# Autodesk Inventor assembly: AviBay
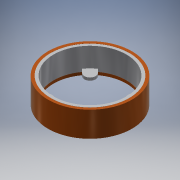
[picture p0: Inventor's stored thumbnail of the model, 180x180]
Saved by Autodesk Inventor 2017 (Build 210142000, 142)
## iProperties
Created: 2016-10-18
Part Number: AviBay
Document SubType Name: Assembly
Designer: cflannery
Author: cflannery
## Documents named in this file (3)
- D:\Triton_Rocket_Club\Propulsion\Launches\8-inch-flight\Design\CAD\Other\AviBay\trunk\AviBay.iam
- D:\Triton_Rocket_Club\Propulsion\Launches\8-inch-flight\Design\CAD\Other\AviBay\trunk\aluminumMount.ipt
- D:\Triton_Rocket_Club\Propulsion\Launches\8-inch-flight\Design\CAD\Other\AviBay\trunk\phenolicLiner.ipt
## Components (2 placed, 2 different names)
1. aluminumMount:1 — Mate:1, Mate:2
2. phenolicLiner:1 — Mate:1, Mate:2
## Relationships (2: Mate 2)
- Mate:1: aluminumMount:1 ↔ phenolicLiner:1
- Mate:2: aluminumMount:1 ↔ phenolicLiner:1
